# Autodesk Inventor assembly: daVinciHead_Sled
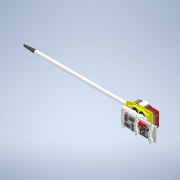
[picture p0: Inventor's stored thumbnail of the model, 180x180]
Saved by Autodesk Inventor 2022 (Build 260153000, 153)
## iProperties
Created: 2022-05-05
Part Number: daVinciHead_Sled
Document SubType Name: Assembly
Designer: 123St
Mass: 527.845 g
Surface Area: 1833.87 cm^2
Volume: 501.873 cm^3
Track2ToolGuidance_Dist: 61,207 mm
Author: 123St
## Documents named in this file (24)
- C:\Users\AEWALDER\Documents\Inventor\03_CurrentProjects\MasterThesis\PSM_V1_Rillenkugellager\Ueberarbeiteter DaVincikopf\daVinciHead_Sled.iam
- C:\Users\AEWALDER\Documents\Inventor\03_CurrentProjects\MasterThesis\PSM_V1_Rillenkugellager\Ueberarbeiteter DaVincikopf\Fuehrungsgrundplatte_V3.ipt
- C:\Users\AEWALDER\Documents\Inventor\03_CurrentProjects\MasterThesis\PSM_V1_Rillenkugellager\Ueberarbeiteter DaVincikopf\JX BLS-HV7146MG.iam
- C:\Users\AEWALDER\Documents\Inventor\03_CurrentProjects\MasterThesis\PSM_V1_Rillenkugellager\Ueberarbeiteter DaVincikopf\Op_dev_gehäuse.ipt
- C:\Users\AEWALDER\Documents\Inventor\03_CurrentProjects\MasterThesis\PSM_V1_Rillenkugellager\Ueberarbeiteter DaVincikopf\Op_dev_stange.ipt
- C:\Users\AEWALDER\Documents\Inventor\03_CurrentProjects\MasterThesis\PSM_V1_Rillenkugellager\Ueberarbeiteter DaVincikopf\Oberteil_servoplatte.ipt
- C:\Users\AEWALDER\Documents\Inventor\03_CurrentProjects\MasterThesis\PSM_V1_Rillenkugellager\ContentCenter\de-DE\ISO 4762(2)\ISO 4762 - M4 x 30ISO.ipt
- C:\Users\AEWALDER\Documents\Inventor\03_CurrentProjects\MasterThesis\PSM_V1_Rillenkugellager\ContentCenter\de-DE\ISO 4762(2)\ISO 4762 - M3 x 12ISO.ipt
- C:\Users\AEWALDER\Documents\Inventor\03_CurrentProjects\MasterThesis\PSM_V1_Rillenkugellager\Ueberarbeiteter DaVincikopf\daVinciTool_Aufnahme.ipt
- C:\Users\AEWALDER\Documents\Inventor\03_CurrentProjects\MasterThesis\PSM_V1_Rillenkugellager\Ueberarbeiteter DaVincikopf\daVinciTool_Aufnahme_ClutchPart.ipt
- C:\Users\AEWALDER\Documents\Inventor\03_CurrentProjects\MasterThesis\PSM_V1_Rillenkugellager\Ueberarbeiteter DaVincikopf\daVincihead_Sled_ToolAufnahmeBuegel.ipt
- C:\Users\AEWALDER\Documents\Inventor\03_CurrentProjects\MasterThesis\PSM_V1_Rillenkugellager\Ueberarbeiteter DaVincikopf\daVincihead_Sled_ToolAufnahmeBuegel_38mm.ipt
- C:\Users\AEWALDER\Documents\Inventor\03_CurrentProjects\MasterThesis\PSM_V1_Rillenkugellager\Ueberarbeiteter DaVincikopf\3mmSchaft_50m.ipt
- C:\Users\AEWALDER\Documents\Inventor\03_CurrentProjects\MasterThesis\PSM_V1_Rillenkugellager\Ueberarbeiteter DaVincikopf\3mmSchaft_63mm.ipt
- C:\Users\AEWALDER\Documents\Inventor\03_CurrentProjects\MasterThesis\PSM_V1_Rillenkugellager\Ueberarbeiteter DaVincikopf\Fuehrungsrollen_Assembly.iam
- C:\Users\AEWALDER\Documents\Inventor\03_CurrentProjects\MasterThesis\PSM_V1_Rillenkugellager\ContentCenter\de-DE\ISO 4762(2)\ISO 4762 - M3 x 10ISO.ipt
- C:\Users\AEWALDER\Documents\Inventor\03_CurrentProjects\MasterThesis\PSM_V1_Rillenkugellager\Maschinenbauteil\spur_gear_1_30_6_6.ipt
- C:\Users\AEWALDER\Documents\Inventor\03_CurrentProjects\MasterThesis\PSM_V1_Rillenkugellager\Ueberarbeiteter DaVincikopf\daVinciHead_HITEC_Assembly.iam
- C:\Users\AEWALDER\Documents\Inventor\03_CurrentProjects\MasterThesis\PSM_V1_Rillenkugellager\Ueberarbeiteter DaVincikopf\Anpresspinns_Assembly.iam
- C:\Users\AEWALDER\Documents\Inventor\03_CurrentProjects\MasterThesis\PSM_V1_Rillenkugellager\ContentCenter\de-DE\ISO 4762(2)\ISO 4762 - M4 x 12ISO.ipt
- C:\Users\AEWALDER\Documents\Inventor\03_CurrentProjects\MasterThesis\PSM_V1_Rillenkugellager\ContentCenter\de-DE\ISO 10642(1)\ISO 10642 - M3 x  8.ipt
- C:\Users\AEWALDER\Documents\Inventor\03_CurrentProjects\MasterThesis\PSM_V1_Rillenkugellager\ContentCenter\en-US\ISO 4762(1)\DIN EN ISO 4762 - M3 x 16.ipt
- C:\Users\AEWALDER\Documents\Inventor\03_CurrentProjects\MasterThesis\PSM_V1_Rillenkugellager\ContentCenter\en-US\ISO 10642(2)\ISO 10642  - M3  x  10.ipt
- C:\Users\AEWALDER\Documents\Inventor\03_CurrentProjects\MasterThesis\PSM_V1_Rillenkugellager\CableHolder.ipt
## Components (47 placed, 23 different names)
1. Fuehrungsgrundplatte_V3:1 — Fluchtend:1, Passend:1, Passend:2, Passend:34, Fluchtend:9, Fluchtend:10, Fluchtend:11, Passend:38, Passend:42, Passend:138, Passend:139, Passend:140, Passend:141, Passend:142, Passend:143, Passend:144, Passend:145, Passend:146, Passend:167, Passend:168, Passend:169, Passend:170, Passend:171, Passend:172, Passend:173, Passend:174, Passend:175, Passend:176, Passend:177, Passend:178, Passend:189, Mate:195, Mate:196, Mate:197, Mate:198, Flush:16
2. JX BLS-HV7146MG:1 [sub-assembly] — Fluchtend:1, Passend:1, Passend:2, Passend:159, Passend:160, Passend:163, Passend:165, Passend:190
3. daVinciHead_HITEC_Assembly:1 [sub-assembly] — Passend:173, Passend:174, Passend:175
4. daVinciHead_HITEC_Assembly:2 [sub-assembly] — Passend:167, Passend:168, Passend:169, Passend:179
5. daVinciHead_HITEC_Assembly:3 [sub-assembly] — Passend:176, Passend:177, Passend:178, Passend:180
6. daVinciHead_HITEC_Assembly:4 [sub-assembly] — Passend:170, Passend:171, Passend:172
7. Op_dev_gehäuse:1 — Drehbar:18, Passend:68, Passend:69, Passend:193
8. Op_dev_stange:1 — Drehbar:18, Passend:70
9. Oberteil_servoplatte:1 — Passend:34, Fluchtend:9, Passend:110, Passend:113, Passend:123, Passend:125, Passend:127, Passend:129, Passend:131, Passend:132, Passend:133, Passend:134, Passend:181, Passend:183, Passend:185, Passend:186
10. ISO 4762 M4 x 30:1 — Passend:38, Passend:163
11. ISO 4762 M4 x 30:3 — Passend:42, Passend:165
12. DIN EN ISO 4762 M3 x 16:2
13. DIN EN ISO 4762 M3 x 16:3
14. DIN EN ISO 4762 M3 x 16:1
15. DIN EN ISO 4762 M3 x 16:4
16. daVinciTool_Aufnahme:1 — Passend:68, Passend:69, Fluchtend:13, Passend:122, Passend:123, Passend:192, Passend:193
17. daVinciTool_Aufnahme_ClutchPart:1 — Fluchtend:13, Passend:179, Passend:180, Passend:182, Passend:184, Passend:187, Passend:188
18. daVincihead_Sled_ToolAufnahmeBuegel:1 — Passend:110, Passend:115, Passend:128, Passend:130, Passend:134, Fluchtend:14, Fluchtend:15
19. daVincihead_Sled_ToolAufnahmeBuegel_38mm:1 — Passend:113, Passend:116, Passend:117, Passend:124, Passend:126, Passend:132, Passend:133
20. 3mmSchaft_50m:1 — Passend:116, Passend:117
21. 3mmSchaft_63mm:1 — Passend:115, Passend:122, Fluchtend:14
22. ISO 4762 M3 x 12:6 — Passend:124, Passend:125
23. ISO 4762 M3 x 12:5 — Passend:126, Passend:127
24. ISO 4762 M3 x 12:7 — Passend:128, Passend:129
25. ISO 4762 M3 x 12:8 — Passend:130, Passend:131
26. Fuehrungsrollen_Assembly:2 [sub-assembly] — Passend:138, Passend:139, Passend:140, Passend:147, Passend:148, Passend:149, Passend:150
27. Fuehrungsrollen_Assembly:3 [sub-assembly] — Passend:141, Passend:142, Passend:143, Passend:151, Passend:152, Passend:153, Passend:154
28. Fuehrungsrollen_Assembly:4 [sub-assembly] — Passend:144, Passend:145, Passend:146, Passend:155, Passend:156, Passend:157, Passend:158, Winkel:3, Tangential:1
29. ISO 4762 M3 x 10:1 — Passend:147, Passend:148
30. ISO 4762 M3 x 10:2 — Passend:149, Passend:150
31. ISO 4762 M3 x 10:3 — Passend:151, Passend:152
32. ISO 4762 M3 x 10:4 — Passend:153, Passend:154
33. ISO 4762 M3 x 10:5 — Passend:155, Passend:156
34. ISO 4762 M3 x 10:6 — Passend:157, Passend:158
35. spur_gear_1_30_6_6:1 — Passend:159, Passend:160, Passend:194
36. Anpresspinns_Assembly:1 [sub-assembly] — Passend:181, Passend:182
37. Anpresspinns_Assembly:2 [sub-assembly] — Passend:183, Passend:184
38. Anpresspinns_Assembly:3 [sub-assembly] — Passend:186, Passend:188
39. Anpresspinns_Assembly:4 [sub-assembly] — Passend:185, Passend:187
40. ISO 4762 M4 x 12:1 — Passend:189, Passend:190
41. 3mmSchaft_63mm:2 — Passend:192, Fluchtend:15
42. ISO 10642 M3x8:1 — Passend:194
43. DIN EN ISO 10642 M3  x  10:1 — Mate:195
44. DIN EN ISO 10642 M3  x  10:2 — Mate:196
45. DIN EN ISO 10642 M3  x  10:3 — Mate:197
46. DIN EN ISO 10642 M3  x  10:4 — Mate:198
47. CableHolder:1 — Flush:16
## Relationships (104: Mate 92, Flush 8, Angle 2, RevoluteJoint 1, Tangent 1)
- Fluchtend:1 [Flush] (-5 mm): Fuehrungsgrundplatte_V3:1 ↔ JX BLS-HV7146MG:1
- Passend:1 [Mate]: Fuehrungsgrundplatte_V3:1 ↔ JX BLS-HV7146MG:1
- Passend:2 [Mate]: Fuehrungsgrundplatte_V3:1 ↔ JX BLS-HV7146MG:1
- Drehbar:18 [RevoluteJoint]: Op_dev_gehäuse:1 ↔ Op_dev_stange:1
- Passend:34 [Mate]: Fuehrungsgrundplatte_V3:1 ↔ Oberteil_servoplatte:1
- Fluchtend:9 [Flush]: Fuehrungsgrundplatte_V3:1 ↔ Oberteil_servoplatte:1
- Fluchtend:10 [Flush]: Fuehrungsgrundplatte_V3:1
- Fluchtend:11 [Flush]: Fuehrungsgrundplatte_V3:1
- Passend:38 [Mate]: Fuehrungsgrundplatte_V3:1 ↔ ISO 4762 M4 x 30:1
- Passend:42 [Mate]: Fuehrungsgrundplatte_V3:1 ↔ ISO 4762 M4 x 30:3
- [Mate]: Oberteil_servoplatte:1 ↔ DIN EN ISO 4762 M3 x 16:2
- [Mate]: Oberteil_servoplatte:1 ↔ DIN EN ISO 4762 M3 x 16:2
- [Mate]: Oberteil_servoplatte:1 ↔ DIN EN ISO 4762 M3 x 16:3
- [Mate]: Oberteil_servoplatte:1 ↔ DIN EN ISO 4762 M3 x 16:3
- [Mate]: Oberteil_servoplatte:1 ↔ DIN EN ISO 4762 M3 x 16:1
- [Mate]: Oberteil_servoplatte:1 ↔ DIN EN ISO 4762 M3 x 16:1
- [Mate]: Oberteil_servoplatte:1 ↔ DIN EN ISO 4762 M3 x 16:4
- [Mate]: Oberteil_servoplatte:1 ↔ DIN EN ISO 4762 M3 x 16:4
- Passend:68 [Mate] (-6.043 mm): Op_dev_gehäuse:1 ↔ daVinciTool_Aufnahme:1
- Passend:69 [Mate]: Op_dev_gehäuse:1 ↔ daVinciTool_Aufnahme:1
- Passend:70 [Mate]: Op_dev_stange:1
- Passend:71 [Mate]
- Winkel:2 [Angle] (0 deg)
- Fluchtend:13 [Flush]: daVinciTool_Aufnahme:1 ↔ daVinciTool_Aufnahme_ClutchPart:1
- Passend:110 [Mate]: Oberteil_servoplatte:1 ↔ daVincihead_Sled_ToolAufnahmeBuegel:1
- Passend:113 [Mate]: Oberteil_servoplatte:1 ↔ daVincihead_Sled_ToolAufnahmeBuegel_38mm:1
- Passend:115 [Mate]: daVincihead_Sled_ToolAufnahmeBuegel:1 ↔ 3mmSchaft_63mm:1
- Passend:116 [Mate]: daVincihead_Sled_ToolAufnahmeBuegel_38mm:1 ↔ 3mmSchaft_50m:1
- Passend:117 [Mate]: daVincihead_Sled_ToolAufnahmeBuegel_38mm:1 ↔ 3mmSchaft_50m:1
- Passend:122 [Mate]: daVinciTool_Aufnahme:1 ↔ 3mmSchaft_63mm:1
- Passend:123 [Mate]: Oberteil_servoplatte:1 ↔ daVinciTool_Aufnahme:1
- Passend:124 [Mate]: daVincihead_Sled_ToolAufnahmeBuegel_38mm:1 ↔ ISO 4762 M3 x 12:6
- Passend:125 [Mate]: Oberteil_servoplatte:1 ↔ ISO 4762 M3 x 12:6
- Passend:126 [Mate]: daVincihead_Sled_ToolAufnahmeBuegel_38mm:1 ↔ ISO 4762 M3 x 12:5
- Passend:127 [Mate]: Oberteil_servoplatte:1 ↔ ISO 4762 M3 x 12:5
- Passend:128 [Mate]: daVincihead_Sled_ToolAufnahmeBuegel:1 ↔ ISO 4762 M3 x 12:7
- Passend:129 [Mate]: Oberteil_servoplatte:1 ↔ ISO 4762 M3 x 12:7
- Passend:130 [Mate]: daVincihead_Sled_ToolAufnahmeBuegel:1 ↔ ISO 4762 M3 x 12:8
- Passend:131 [Mate]: Oberteil_servoplatte:1 ↔ ISO 4762 M3 x 12:8
- Passend:132 [Mate]: Oberteil_servoplatte:1 ↔ daVincihead_Sled_ToolAufnahmeBuegel_38mm:1
- Passend:133 [Mate]: Oberteil_servoplatte:1 ↔ daVincihead_Sled_ToolAufnahmeBuegel_38mm:1
- Passend:134 [Mate]: Oberteil_servoplatte:1 ↔ daVincihead_Sled_ToolAufnahmeBuegel:1
- Passend:138 [Mate]: Fuehrungsgrundplatte_V3:1 ↔ Fuehrungsrollen_Assembly:2
- Passend:139 [Mate]: Fuehrungsgrundplatte_V3:1 ↔ Fuehrungsrollen_Assembly:2
- Passend:140 [Mate]: Fuehrungsgrundplatte_V3:1 ↔ Fuehrungsrollen_Assembly:2
- Passend:141 [Mate]: Fuehrungsgrundplatte_V3:1 ↔ Fuehrungsrollen_Assembly:3
- Passend:142 [Mate]: Fuehrungsgrundplatte_V3:1 ↔ Fuehrungsrollen_Assembly:3
- Passend:143 [Mate]: Fuehrungsgrundplatte_V3:1 ↔ Fuehrungsrollen_Assembly:3
- Passend:144 [Mate]: Fuehrungsgrundplatte_V3:1 ↔ Fuehrungsrollen_Assembly:4
- Passend:145 [Mate]: Fuehrungsgrundplatte_V3:1 ↔ Fuehrungsrollen_Assembly:4
- Passend:146 [Mate]: Fuehrungsgrundplatte_V3:1 ↔ Fuehrungsrollen_Assembly:4
- Passend:147 [Mate]: Fuehrungsrollen_Assembly:2 ↔ ISO 4762 M3 x 10:1
- Passend:148 [Mate]: Fuehrungsrollen_Assembly:2 ↔ ISO 4762 M3 x 10:1
- Passend:149 [Mate]: Fuehrungsrollen_Assembly:2 ↔ ISO 4762 M3 x 10:2
- Passend:150 [Mate]: Fuehrungsrollen_Assembly:2 ↔ ISO 4762 M3 x 10:2
- Passend:151 [Mate]: Fuehrungsrollen_Assembly:3 ↔ ISO 4762 M3 x 10:3
- Passend:152 [Mate]: Fuehrungsrollen_Assembly:3 ↔ ISO 4762 M3 x 10:3
- Passend:153 [Mate]: Fuehrungsrollen_Assembly:3 ↔ ISO 4762 M3 x 10:4
- Passend:154 [Mate]: Fuehrungsrollen_Assembly:3 ↔ ISO 4762 M3 x 10:4
- Passend:155 [Mate]: Fuehrungsrollen_Assembly:4 ↔ ISO 4762 M3 x 10:5
- Passend:156 [Mate]: Fuehrungsrollen_Assembly:4 ↔ ISO 4762 M3 x 10:5
- Passend:157 [Mate]: Fuehrungsrollen_Assembly:4 ↔ ISO 4762 M3 x 10:6
- Passend:158 [Mate]: Fuehrungsrollen_Assembly:4 ↔ ISO 4762 M3 x 10:6
- Passend:159 [Mate]: JX BLS-HV7146MG:1 ↔ spur_gear_1_30_6_6:1
- Passend:160 [Mate]: JX BLS-HV7146MG:1 ↔ spur_gear_1_30_6_6:1
- Passend:163 [Mate]: JX BLS-HV7146MG:1 ↔ ISO 4762 M4 x 30:1
- Passend:165 [Mate]: JX BLS-HV7146MG:1 ↔ ISO 4762 M4 x 30:3
- Winkel:3 [Angle] (0 deg): Fuehrungsrollen_Assembly:4
- Tangential:1: Fuehrungsrollen_Assembly:4
- Passend:167 [Mate]: Fuehrungsgrundplatte_V3:1 ↔ daVinciHead_HITEC_Assembly:2
- Passend:168 [Mate]: Fuehrungsgrundplatte_V3:1 ↔ daVinciHead_HITEC_Assembly:2
- Passend:169 [Mate]: Fuehrungsgrundplatte_V3:1 ↔ daVinciHead_HITEC_Assembly:2
- Passend:170 [Mate]: Fuehrungsgrundplatte_V3:1 ↔ daVinciHead_HITEC_Assembly:4
- Passend:171 [Mate]: Fuehrungsgrundplatte_V3:1 ↔ daVinciHead_HITEC_Assembly:4
- Passend:172 [Mate]: Fuehrungsgrundplatte_V3:1 ↔ daVinciHead_HITEC_Assembly:4
- Passend:173 [Mate]: Fuehrungsgrundplatte_V3:1 ↔ daVinciHead_HITEC_Assembly:1
- Passend:174 [Mate]: Fuehrungsgrundplatte_V3:1 ↔ daVinciHead_HITEC_Assembly:1
- Passend:175 [Mate]: Fuehrungsgrundplatte_V3:1 ↔ daVinciHead_HITEC_Assembly:1
- Passend:176 [Mate]: Fuehrungsgrundplatte_V3:1 ↔ daVinciHead_HITEC_Assembly:3
- Passend:177 [Mate]: Fuehrungsgrundplatte_V3:1 ↔ daVinciHead_HITEC_Assembly:3
- Passend:178 [Mate]: Fuehrungsgrundplatte_V3:1 ↔ daVinciHead_HITEC_Assembly:3
- Passend:179 [Mate]: daVinciHead_HITEC_Assembly:2 ↔ daVinciTool_Aufnahme_ClutchPart:1
- Passend:180 [Mate]: daVinciHead_HITEC_Assembly:3 ↔ daVinciTool_Aufnahme_ClutchPart:1
- Passend:181 [Mate]: Oberteil_servoplatte:1 ↔ Anpresspinns_Assembly:1
- Passend:182 [Mate]: daVinciTool_Aufnahme_ClutchPart:1 ↔ Anpresspinns_Assembly:1
- Passend:183 [Mate]: Oberteil_servoplatte:1 ↔ Anpresspinns_Assembly:2
- Passend:184 [Mate]: daVinciTool_Aufnahme_ClutchPart:1 ↔ Anpresspinns_Assembly:2
- Passend:185 [Mate]: Oberteil_servoplatte:1 ↔ Anpresspinns_Assembly:4
- Passend:186 [Mate]: Oberteil_servoplatte:1 ↔ Anpresspinns_Assembly:3
- Passend:187 [Mate]: daVinciTool_Aufnahme_ClutchPart:1 ↔ Anpresspinns_Assembly:4
- Passend:188 [Mate]: daVinciTool_Aufnahme_ClutchPart:1 ↔ Anpresspinns_Assembly:3
- Passend:189 [Mate]: Fuehrungsgrundplatte_V3:1 ↔ ISO 4762 M4 x 12:1
- Passend:190 [Mate]: JX BLS-HV7146MG:1 ↔ ISO 4762 M4 x 12:1
- [Mate]: Fuehrungsgrundplatte_V3:1 ↔ DIN EN ISO 4762 M3 x 16:2
- Fluchtend:14 [Flush]: daVincihead_Sled_ToolAufnahmeBuegel:1 ↔ 3mmSchaft_63mm:1
- Passend:192 [Mate]: daVinciTool_Aufnahme:1 ↔ 3mmSchaft_63mm:2
- Fluchtend:15 [Flush]: daVincihead_Sled_ToolAufnahmeBuegel:1 ↔ 3mmSchaft_63mm:2
- Passend:193 [Mate]: Op_dev_gehäuse:1 ↔ daVinciTool_Aufnahme:1
- Passend:194 [Mate]: spur_gear_1_30_6_6:1 ↔ ISO 10642 M3x8:1
- Mate:195: Fuehrungsgrundplatte_V3:1 ↔ DIN EN ISO 10642 M3  x  10:1
- Mate:196: Fuehrungsgrundplatte_V3:1 ↔ DIN EN ISO 10642 M3  x  10:2
- Mate:197: Fuehrungsgrundplatte_V3:1 ↔ DIN EN ISO 10642 M3  x  10:3
- Mate:198: Fuehrungsgrundplatte_V3:1 ↔ DIN EN ISO 10642 M3  x  10:4
- Flush:16: Fuehrungsgrundplatte_V3:1 ↔ CableHolder:1
## Named parameters: Track2ToolGuidance_Dist = 61.20692 mm
